# Autodesk Inventor assembly: MIRarmアーム先端
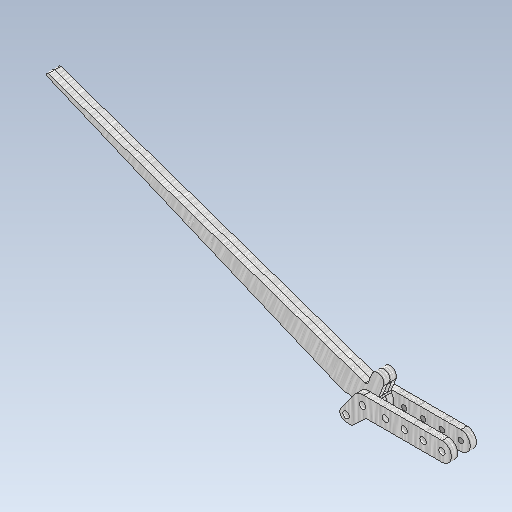
[picture p0: Inventor's stored thumbnail of the model, 512x512]
Saved by Autodesk Inventor 2020.2 (Build 242310000, 310)
## iProperties
Created: 2020-03-28
Part Number: MIRarmアーム先端
Document SubType Name: Assembly
Designer: aoyama
Mass: 25.9087 g
Surface Area: 109.67 cm^2
Volume: 9.28611 cm^3
Density: 2.79005 g/cm^3
Author: aoyam
## Documents named in this file (7)
- C:\Users\aoyam\Desktop\SRDC_local\Inventor\二年機\Geminiβ\腕\MIR達\MIRarmアーム先端.iam
- C:\Users\aoyam\Desktop\SRDC_local\Inventor\二年機\Geminiβ\腕\MIR達\MIRarm中間節アーム先端締結パーツipt.ipt
- C:\Users\aoyam\Desktop\SRDC_local\Inventor\二年機\Geminiβ\腕\MIR達\MIRarmアーム先端.ipt
- C:\Users\aoyam\Desktop\SRDC_local\Inventor\二年機\Geminiβ\汎用部品\MIR達\MIRarmスペーサー中空M3L6アルミ.ipt
- C:\Users\aoyam\Desktop\SRDC_local\Inventor\二年機\Geminiβ\汎用部品\MIR達\MIRarmオイレスd6D8L6.ipt
- C:\Users\aoyam\Desktop\SRDC_local\Inventor\二年機\Geminiβ\腕\中間節アーム先端締結パーツ外.ipt
- C:\Users\aoyam\Desktop\SRDC_local\Inventor\二年機\Geminiβ\腕\MIR達\MIRMIRarmアーム先端.ipt
## Components (7 placed, 6 different names)
1. MIRarm中間節アーム先端締結パーツipt:2 — 挿入:5, 挿入:8
2. MIRarmアーム先端:2 — 挿入:12, 挿入:13, フラッシュ:1
3. MIRarmスペーサー中空M3L6アルミ:1 — 挿入:8, 挿入:10
4. MIRarmスペーサー中空M3L6アルミ:2 — 挿入:5, 挿入:9, 挿入:11
5. MIRarmオイレスd6D8L6:1 — 挿入:11, 挿入:12
6. 中間節アーム先端締結パーツ外:1 — 挿入:9, 挿入:10
7. MIRMIRarmアーム先端:1 — 挿入:13, フラッシュ:1
## Relationships (8: Insert 7, Flush 1)
- 挿入:5 [Insert]: MIRarm中間節アーム先端締結パーツipt:2 ↔ MIRarmスペーサー中空M3L6アルミ:2
- 挿入:8 [Insert]: MIRarm中間節アーム先端締結パーツipt:2 ↔ MIRarmスペーサー中空M3L6アルミ:1
- 挿入:9 [Insert]: MIRarmスペーサー中空M3L6アルミ:2 ↔ 中間節アーム先端締結パーツ外:1
- 挿入:10 [Insert]: MIRarmスペーサー中空M3L6アルミ:1 ↔ 中間節アーム先端締結パーツ外:1
- 挿入:11 [Insert]: MIRarmスペーサー中空M3L6アルミ:2 ↔ MIRarmオイレスd6D8L6:1
- 挿入:12 [Insert]: MIRarmアーム先端:2 ↔ MIRarmオイレスd6D8L6:1
- 挿入:13 [Insert]: MIRarmアーム先端:2 ↔ MIRMIRarmアーム先端:1
- フラッシュ:1 [Flush]: MIRarmアーム先端:2 ↔ MIRMIRarmアーム先端:1
